# Autodesk Inventor assembly: FrameAssembly
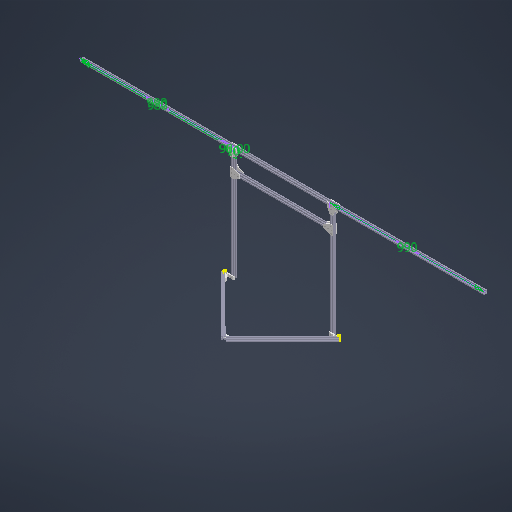
[picture p0: Inventor's stored thumbnail of the model, 512x512]
Saved by Autodesk Inventor 2026 (Build 300175050, 175E)
## iProperties
Created: 2025-06-09
Part Number: FrameAssembly
Document SubType Name: Assembly
Designer: aadit
Author: aadit
## Documents named in this file (14)
- C:\Users\aadit\OneDrive\Documents\GitHub\SWIFT-UAV\System_development\Pelican\v0.2\SubAssemblies\FrameAssembly\FrameAssembly.iam
- C:\Users\aadit\Downloads\CAD stuff\3842517173_3D_214\3842517173_3D_214\3842517173_3D_214.ipt
- C:\Users\aadit\OneDrive\Documents\GitHub\SWIFT-UAV\System_development\Pelican\v0.2\SubAssemblies\FrameAssembly\Parts\2020 T Plate Bracket Connectors .ipt
- C:\Users\aadit\OneDrive\Documents\GitHub\SWIFT-UAV\System_development\Pelican\v0.2\SubAssemblies\FrameAssembly\Parts\8020-14122\8020-14122\8020-14122.ipt
- C:\Users\aadit\OneDrive\Documents\Inventor\Content Center Files\R2026\en-US\AS 1237 (2.1)\AS 1237 - 4.ipt
- C:\Users\aadit\Documents\Inventor\Content Center Files\R2026\en-US\DIN 6912\DIN 6912 - M4 x 10.ipt
- C:\Users\aadit\OneDrive\Documents\GitHub\SWIFT-UAV\System_development\Pelican\v0.2\SubAssemblies\FrameAssembly\Parts\STRUT PROFILE 20X20 L=3100\STRUT PROFILE 20X20 L=3100\STRUT PROFILE 20X20 L=3100.ipt
- C:\Users\aadit\OneDrive\Documents\GitHub\SWIFT-UAV\System_development\Pelican\v0.2\SubAssemblies\FrameAssembly\Parts\20 Series 2 Hole - 18mm Slotted Inside Corner Bracket with Dual Support\20 Series 2 Hole - 18.ipt
- C:\Users\aadit\OneDrive\Documents\Inventor\Content Center Files\R2026\en-US\AS 1237 (2.1)\AS 1237 - 5.ipt
- C:\Users\aadit\OneDrive\Documents\Inventor\Content Center Files\R2026\en-US\DIN 6912\DIN 6912 - M5 x 16.ipt
- C:\Users\aadit\OneDrive\Documents\Inventor\Content Center Files\R2026\en-US\DIN 6912\DIN 6912 - M5 x 12.ipt
- C:\Users\aadit\OneDrive\Documents\Inventor\Content Center Files\R2026\en-US\DIN 6912\DIN 6912 - M4 x 12.ipt
- C:\Users\aadit\OneDrive\Documents\GitHub\SWIFT-UAV\System_development\Pelican\v0.2\SubAssemblies\FrameAssembly\Parts\45 Degree Connector .ipt
- C:\Users\aadit\OneDrive\Documents\GitHub\SWIFT-UAV\System_development\Pelican\v0.2\SubAssemblies\FrameAssembly\Parts\T-Nut Block\T-Nut Block\T-Nut Block.ipt
## Components (239 placed, 13 different names)
1. 3842517173_3D_214:1 — Flush:2, Mate:1, Flush:3, Flush:4, Flush:5, Flush:6, Flush:7, Flush:8, Flush:9, Flush:10, Mate:52, Mate:53, Mate:54, Mate:55
2. 3842517173_3D_214:4 — Mate:1, Flush:3, Flush:4, Flush:5, Flush:6, Flush:11, Flush:12, Flush:15, Flush:16, Mate:49, Mate:51, Mate:60, Mate:63, Mate:64
3. 3842517173_3D_214:5 — Flush:2, Flush:13, Flush:14, Flush:17, Flush:18, Mate:48, Mate:50, Mate:58, Mate:59, Mate:61, Mate:62, Mate:67
4. 2020 T Plate Bracket Connectors :1 — Flush:7, Mate:2, Mate:3, Mate:4, Mate:5, Mate:6, Insert:1, Insert:2, Insert:3, Insert:4, Insert:5, Insert:6, Insert:7, Insert:8, Insert:9, Insert:10
5. 2020 T Plate Bracket Connectors :2 — Flush:8, Mate:7, Mate:8, Mate:9, Mate:10, Mate:11, Insert:14, Insert:15, Insert:16, Insert:17, Insert:18, Insert:19, Insert:20, Insert:21, Insert:22
6. 2020 T Plate Bracket Connectors :5 — Flush:10, Mate:17, Mate:18, Mate:19, Mate:20, Mate:21, Insert:28, Insert:29, Insert:30, Insert:31, Insert:32, Insert:33, Insert:34, Insert:35, Insert:36, Insert:39
7. 2020 T Plate Bracket Connectors :8 — Flush:9, Mate:12, Mate:13, Mate:14, Mate:15, Mate:16, Mate:22, Mate:23, Mate:24, Mate:25, Mate:26, Insert:42, Insert:43, Insert:44, Insert:45, Insert:46, Insert:47, Insert:48, Insert:49, Insert:50
8. 8020-14122:1 — Mate:2
9. 8020-14122:2 — Mate:3
10. 8020-14122:3 — Mate:4
11. 8020-14122:4 — Mate:5
12. 8020-14122:5 — Mate:6
13. 8020-14122:6 — Mate:7
14. AS 1237 (2.1) 4:1 — Insert:1
15. AS 1237 (2.1) 4:2 — Insert:2
16. AS 1237 (2.1) 4:3 — Insert:3
17. AS 1237 (2.1) 4:4 — Insert:4
18. AS 1237 (2.1) 4:5 — Insert:5
19. AS 1237 (2.1) 4:6 — Insert:6, Insert:11
20. AS 1237 (2.1) 4:7 — Insert:7, Insert:12
21. AS 1237 (2.1) 4:8 — Insert:8, Insert:13
22. AS 1237 (2.1) 4:9 — Insert:9, Insert:151
23. DIN 6912 M4 x 10:1 — Insert:10
24. DIN 6912 M4 x 10:2 — Insert:11
25. DIN 6912 M4 x 10:3 — Insert:12
26. DIN 6912 M4 x 10:4 — Insert:13
27. 8020-14122:7 — Mate:8
28. 8020-14122:8 — Mate:9
29. 8020-14122:9 — Mate:10
30. 8020-14122:10 — Mate:32
31. 8020-14122:11 — Mate:11
32. AS 1237 (2.1) 4:10 — Insert:14, Insert:132
33. AS 1237 (2.1) 4:11 — Insert:15, Insert:23
34. AS 1237 (2.1) 4:12 — Insert:16
35. AS 1237 (2.1) 4:13 — Insert:17
36. AS 1237 (2.1) 4:14 — Insert:18
37. AS 1237 (2.1) 4:15 — Insert:19, Insert:24
38. AS 1237 (2.1) 4:16 — Insert:20, Insert:25
39. AS 1237 (2.1) 4:17 — Insert:21, Insert:26
40. AS 1237 (2.1) 4:18 — Insert:22, Insert:27
41. DIN 6912 M4 x 10:5 — Insert:23
42. DIN 6912 M4 x 10:6 — Insert:24
43. DIN 6912 M4 x 10:7 — Insert:25
44. DIN 6912 M4 x 10:8 — Insert:26
45. DIN 6912 M4 x 10:9 — Insert:27
46. 8020-14122:12 — Mate:12
47. 8020-14122:13 — Mate:13
48. 8020-14122:14 — Mate:14
49. 8020-14122:15 — Mate:16
50. 8020-14122:16 — Mate:15
51. 8020-14122:17 — Mate:17
52. 8020-14122:18 — Mate:19
53. 8020-14122:19 — Mate:21
54. 8020-14122:20 — Mate:18
55. 8020-14122:21 — Mate:20
56. AS 1237 (2.1) 4:19 — Insert:28, Insert:37
57. AS 1237 (2.1) 4:20 — Insert:29
58. AS 1237 (2.1) 4:21 — Insert:30
59. AS 1237 (2.1) 4:22 — Insert:31
60. AS 1237 (2.1) 4:23 — Insert:32
61. AS 1237 (2.1) 4:24 — Insert:33, Insert:38
62. AS 1237 (2.1) 4:25 — Insert:34
63. AS 1237 (2.1) 4:26 — Insert:35, Insert:40
64. AS 1237 (2.1) 4:27 — Insert:36, Insert:41
65. DIN 6912 M4 x 10:10 — Insert:37
66. DIN 6912 M4 x 10:11 — Insert:38
67. DIN 6912 M4 x 10:12 — Insert:39
68. DIN 6912 M4 x 10:13 — Insert:40
69. DIN 6912 M4 x 10:14 — Insert:41
70. 8020-14122:22 — Mate:23
71. 8020-14122:23 — Mate:22
72. 8020-14122:24 — Mate:24
73. 8020-14122:25 — Mate:25
74. 8020-14122:26 — Mate:26
75. AS 1237 (2.1) 4:28 — Insert:42, Insert:150
76. AS 1237 (2.1) 4:29 — Insert:43
77. AS 1237 (2.1) 4:30 — Insert:44
78. AS 1237 (2.1) 4:31 — Insert:45
79. AS 1237 (2.1) 4:32 — Insert:46, Insert:51
80. AS 1237 (2.1) 4:33 — Insert:47, Insert:52
81. AS 1237 (2.1) 4:34 — Insert:48, Insert:54
82. AS 1237 (2.1) 4:35 — Insert:49, Insert:53
83. AS 1237 (2.1) 4:36 — Insert:50, Insert:55
84. DIN 6912 M4 x 10:15 — Insert:51
85. DIN 6912 M4 x 10:16 — Insert:52
86. DIN 6912 M4 x 10:17 — Insert:53
87. DIN 6912 M4 x 10:18 — Insert:54
88. DIN 6912 M4 x 10:19 — Insert:55
89. STRUT PROFILE 20X20 L=3100:1 — Flush:11, Flush:12, Flush:13, Flush:14, Mate:57
90. 2020 T Plate Bracket Connectors :9 — Flush:15, Mate:43, Mate:44, Mate:45, Mate:46, Mate:47, Insert:98, Insert:99, Insert:100, Insert:101, Insert:102, Insert:103, Insert:104, Insert:105, Insert:106
91. 2020 T Plate Bracket Connectors :10 — Flush:16, Mate:33, Mate:34, Mate:35, Mate:36, Mate:37, Insert:70, Insert:71, Insert:72, Insert:73, Insert:74, Insert:75, Insert:76, Insert:77, Insert:78
92. 2020 T Plate Bracket Connectors :11 — Flush:17, Mate:38, Mate:39, Mate:40, Mate:41, Mate:42, Insert:84, Insert:85, Insert:86, Insert:87, Insert:88, Insert:89, Insert:90, Insert:91, Insert:92
93. 2020 T Plate Bracket Connectors :12 — Flush:18, Mate:27, Mate:28, Mate:29, Mate:30, Mate:31, Mate:32, Insert:56, Insert:57, Insert:58, Insert:59, Insert:60, Insert:61, Insert:62, Insert:63, Insert:64, Insert:65
94. 8020-14122:28 — Mate:27
95. 8020-14122:29 — Mate:30
96. 8020-14122:30 — Mate:28
97. 8020-14122:31 — Mate:31
98. 8020-14122:32 — Mate:29
99. 8020-14122:33 — Mate:51, Insert:126, Insert:127
100. AS 1237 (2.1) 4:37 — Insert:56
101. AS 1237 (2.1) 4:38 — Insert:57
102. AS 1237 (2.1) 4:39 — Insert:58
103. AS 1237 (2.1) 4:40 — Insert:59
104. AS 1237 (2.1) 4:41 — Insert:60
105. AS 1237 (2.1) 4:42 — Insert:61, Insert:66
106. AS 1237 (2.1) 4:43 — Insert:62, Insert:68
107. AS 1237 (2.1) 4:44 — Insert:63, Insert:67
108. AS 1237 (2.1) 4:45 — Insert:64, Insert:69
109. DIN 6912 M4 x 10:20 — Insert:65
110. DIN 6912 M4 x 10:21 — Insert:66
111. DIN 6912 M4 x 10:22 — Insert:67
112. DIN 6912 M4 x 10:23 — Insert:68
113. DIN 6912 M4 x 10:24 — Insert:69
114. 8020-14122:41 — Mate:33
115. 8020-14122:42 — Mate:35
116. 8020-14122:43 — Mate:34
117. 8020-14122:44 — Mate:36
118. 8020-14122:45 — Mate:37
119. AS 1237 (2.1) 4:46 — Insert:70, Insert:149
120. AS 1237 (2.1) 4:47 — Insert:71, Insert:79
121. AS 1237 (2.1) 4:48 — Insert:72
122. AS 1237 (2.1) 4:49 — Insert:73
123. AS 1237 (2.1) 4:50 — Insert:74
124. AS 1237 (2.1) 4:51 — Insert:75, Insert:80
125. AS 1237 (2.1) 4:52 — Insert:76, Insert:81
126. AS 1237 (2.1) 4:53 — Insert:77, Insert:82
127. AS 1237 (2.1) 4:54 — Insert:78, Insert:83
128. DIN 6912 M4 x 10:25 — Insert:79
129. DIN 6912 M4 x 10:26 — Insert:80
130. DIN 6912 M4 x 10:27 — Insert:81
131. DIN 6912 M4 x 10:28 — Insert:82
132. DIN 6912 M4 x 10:29 — Insert:83
133. 8020-14122:46 — Mate:39
134. 8020-14122:47 — Mate:40
135. 8020-14122:48 — Mate:41
136. 8020-14122:49 — Mate:42
137. 8020-14122:50 — Mate:38
138. AS 1237 (2.1) 4:55 — Insert:84, Insert:148
139. AS 1237 (2.1) 4:56 — Insert:85, Insert:93
140. AS 1237 (2.1) 4:57 — Insert:86
141. AS 1237 (2.1) 4:58 — Insert:87
142. AS 1237 (2.1) 4:59 — Insert:88
143. AS 1237 (2.1) 4:60 — Insert:89, Insert:94
144. AS 1237 (2.1) 4:61 — Insert:90, Insert:95
145. AS 1237 (2.1) 4:62 — Insert:91, Insert:96
146. AS 1237 (2.1) 4:63 — Insert:92, Insert:97
147. DIN 6912 M4 x 10:30 — Insert:93
148. DIN 6912 M4 x 10:31 — Insert:94
149. DIN 6912 M4 x 10:32 — Insert:95
150. DIN 6912 M4 x 10:33 — Insert:96
151. DIN 6912 M4 x 10:34 — Insert:97
152. 8020-14122:51 — Mate:47
153. 8020-14122:52 — Mate:43
154. 8020-14122:53 — Mate:46
155. 8020-14122:54 — Mate:44
156. 8020-14122:55 — Mate:45
157. AS 1237 (2.1) 4:64 — Insert:98, Insert:107
158. AS 1237 (2.1) 4:65 — Insert:99
159. AS 1237 (2.1) 4:66 — Insert:100
160. AS 1237 (2.1) 4:67 — Insert:101
161. AS 1237 (2.1) 4:68 — Insert:102
162. AS 1237 (2.1) 4:69 — Insert:103, Insert:108
163. AS 1237 (2.1) 4:70 — Insert:104, Insert:109
164. AS 1237 (2.1) 4:71 — Insert:105, Insert:110
165. AS 1237 (2.1) 4:72 — Insert:106, Insert:111
166. DIN 6912 M4 x 10:35 — Insert:107
167. DIN 6912 M4 x 10:36 — Insert:108
168. DIN 6912 M4 x 10:37 — Insert:109
169. DIN 6912 M4 x 10:38 — Insert:110
170. DIN 6912 M4 x 10:39 — Insert:111
171. 20 Series 2 Hole - 18:12
172. 20 Series 2 Hole - 18:14
173. 8020-14122:56 — Mate:48, Insert:112, Insert:113
174. 8020-14122:57 — Mate:49, Insert:122, Insert:123
175. 8020-14122:58 — Mate:50, Insert:118, Insert:119
176. 8020-14122:60 — Mate:52, Insert:128, Insert:129
177. 8020-14122:61 — Mate:57, Insert:139, Insert:140, Insert:146
178. 8020-14122:63 — Mate:54, Insert:116, Insert:117, Insert:120
179. 8020-14122:64 — Mate:53, Insert:114, Insert:115, Insert:134
180. 8020-14122:65 — Mate:55, Insert:124, Insert:125
181. AS 1237 (2.1) 5:1 — Insert:112, Insert:133
182. AS 1237 (2.1) 5:2 — Insert:113
183. AS 1237 (2.1) 5:3 — Insert:114
184. AS 1237 (2.1) 5:4 — Insert:115
185. AS 1237 (2.1) 5:5 — Insert:116
186. AS 1237 (2.1) 5:6 — Insert:117
187. AS 1237 (2.1) 5:7 — Insert:118
188. AS 1237 (2.1) 5:8 — Insert:119, Insert:135
189. AS 1237 (2.1) 5:9 — Insert:120, Insert:136
190. AS 1237 (2.1) 5:11 — Insert:122, Insert:147
191. AS 1237 (2.1) 5:12 — Insert:123
192. AS 1237 (2.1) 5:13 — Insert:124
193. AS 1237 (2.1) 5:14 — Insert:125, Insert:131
194. AS 1237 (2.1) 5:15 — Insert:126, Insert:137
195. AS 1237 (2.1) 5:16 — Insert:127
196. AS 1237 (2.1) 5:17 — Insert:128
197. AS 1237 (2.1) 5:18 — Insert:129, Insert:138
198. DIN 6912 M5 x 16:2 — Insert:131
199. DIN 6912 M4 x 10:40 — Insert:132
200. DIN 6912 M5 x 12:1 — Insert:133
201. DIN 6912 M4 x 12:1 — Insert:134
202. DIN 6912 M5 x 12:2 — Insert:135
203. DIN 6912 M5 x 12:3 — Insert:136
204. DIN 6912 M5 x 12:4 — Insert:137
205. DIN 6912 M5 x 12:5 — Insert:138
206. 20 Series 2 Hole - 18:16 — Mate:58
207. 8020-14122:67 — Mate:59, Insert:141, Insert:142, Insert:143, Insert:144
208. AS 1237 (2.1) 5:19 — Insert:139
209. AS 1237 (2.1) 5:20 — Insert:140
210. AS 1237 (2.1) 5:21 — Insert:141
211. AS 1237 (2.1) 5:22 — Insert:142
212. AS 1237 (2.1) 5:23 — Insert:143
213. AS 1237 (2.1) 5:24 — Insert:144, Insert:145
214. DIN 6912 M5 x 12:6 — Insert:145
215. DIN 6912 M4 x 12:2 — Insert:146
216. 20 Series 2 Hole - 18:21 — Mate:60
217. 20 Series 2 Hole - 18:22 — Mate:61
218. 20 Series 2 Hole - 18:23 — Mate:62
219. 20 Series 2 Hole - 18:24 — Mate:63
220. DIN 6912 M5 x 12:7 — Insert:147
221. DIN 6912 M4 x 10:41 — Insert:148
222. DIN 6912 M4 x 10:42 — Insert:149
223. DIN 6912 M4 x 10:43 — Insert:150
224. DIN 6912 M4 x 10:44 — Insert:151
225. 45 Degree Connector :1 — Mate:65, Mate:66, Flush:21
226. T-Nut Block:1 — Mate:64
227. T-Nut Block:3 — Mate:67
228. DIN 6912 M4 x 10:45 — Mate:65, Mate:66
229. 45 Degree Connector :2 — Insert:152, Flush:22
230. DIN 6912 M4 x 10:46 — Insert:152
231. STRUT PROFILE 20X20 L=3100:2 — Flush:21, Mate:68
232. STRUT PROFILE 20X20 L=3100:3 — Flush:22, Mate:69
233. 20 Series 2 Hole - 18:25
234. T-Nut Block:4 — Mate:68, Insert:153, Insert:154
235. T-Nut Block:5 — Mate:69, Insert:155, Insert:156
236. DIN 6912 M4 x 10:47 — Insert:153
237. DIN 6912 M4 x 10:48 — Insert:154
238. DIN 6912 M4 x 10:49 — Insert:155
239. DIN 6912 M4 x 10:50 — Insert:156
## Relationships (241: Insert 154, Mate 68, Flush 19)
- Flush:2: 3842517173_3D_214:1 ↔ 3842517173_3D_214:5
- Mate:1: 3842517173_3D_214:1 ↔ 3842517173_3D_214:4
- Flush:3: 3842517173_3D_214:1 ↔ 3842517173_3D_214:4
- Flush:4: 3842517173_3D_214:1 ↔ 3842517173_3D_214:4
- Flush:5: 3842517173_3D_214:1 ↔ 3842517173_3D_214:4
- Flush:6: 3842517173_3D_214:1 ↔ 3842517173_3D_214:4
- Flush:7: 3842517173_3D_214:1 ↔ 2020 T Plate Bracket Connectors :1
- Mate:2: 2020 T Plate Bracket Connectors :1 ↔ 8020-14122:1
- Mate:3: 2020 T Plate Bracket Connectors :1 ↔ 8020-14122:2
- Mate:4: 2020 T Plate Bracket Connectors :1 ↔ 8020-14122:3
- Mate:5: 2020 T Plate Bracket Connectors :1 ↔ 8020-14122:4
- Mate:6: 2020 T Plate Bracket Connectors :1 ↔ 8020-14122:5
- Insert:1: 2020 T Plate Bracket Connectors :1 ↔ AS 1237 (2.1) 4:1
- Insert:2: 2020 T Plate Bracket Connectors :1 ↔ AS 1237 (2.1) 4:2
- Insert:3: 2020 T Plate Bracket Connectors :1 ↔ AS 1237 (2.1) 4:3
- Insert:4: 2020 T Plate Bracket Connectors :1 ↔ AS 1237 (2.1) 4:4
- Insert:5: 2020 T Plate Bracket Connectors :1 ↔ AS 1237 (2.1) 4:5
- Insert:6: 2020 T Plate Bracket Connectors :1 ↔ AS 1237 (2.1) 4:6
- Insert:7: 2020 T Plate Bracket Connectors :1 ↔ AS 1237 (2.1) 4:7
- Insert:8: 2020 T Plate Bracket Connectors :1 ↔ AS 1237 (2.1) 4:8
- Insert:9: 2020 T Plate Bracket Connectors :1 ↔ AS 1237 (2.1) 4:9
- Insert:10: 2020 T Plate Bracket Connectors :1 ↔ DIN 6912 M4 x 10:1
- Insert:11: AS 1237 (2.1) 4:6 ↔ DIN 6912 M4 x 10:2
- Insert:12: AS 1237 (2.1) 4:7 ↔ DIN 6912 M4 x 10:3
- Insert:13: AS 1237 (2.1) 4:8 ↔ DIN 6912 M4 x 10:4
- Flush:8: 3842517173_3D_214:1 ↔ 2020 T Plate Bracket Connectors :2
- Mate:7: 2020 T Plate Bracket Connectors :2 ↔ 8020-14122:6
- Mate:8: 2020 T Plate Bracket Connectors :2 ↔ 8020-14122:7
- Mate:9: 2020 T Plate Bracket Connectors :2 ↔ 8020-14122:8
- Mate:10: 2020 T Plate Bracket Connectors :2 ↔ 8020-14122:9
- Mate:11: 2020 T Plate Bracket Connectors :2 ↔ 8020-14122:11
- Insert:14: 2020 T Plate Bracket Connectors :2 ↔ AS 1237 (2.1) 4:10
- Insert:15: 2020 T Plate Bracket Connectors :2 ↔ AS 1237 (2.1) 4:11
- Insert:16: 2020 T Plate Bracket Connectors :2 ↔ AS 1237 (2.1) 4:12
- Insert:17: 2020 T Plate Bracket Connectors :2 ↔ AS 1237 (2.1) 4:13
- Insert:18: 2020 T Plate Bracket Connectors :2 ↔ AS 1237 (2.1) 4:14
- Insert:19: 2020 T Plate Bracket Connectors :2 ↔ AS 1237 (2.1) 4:15
- Insert:20: 2020 T Plate Bracket Connectors :2 ↔ AS 1237 (2.1) 4:16
- Insert:21: 2020 T Plate Bracket Connectors :2 ↔ AS 1237 (2.1) 4:17
- Insert:22: 2020 T Plate Bracket Connectors :2 ↔ AS 1237 (2.1) 4:18
- Insert:23: AS 1237 (2.1) 4:11 ↔ DIN 6912 M4 x 10:5
- Insert:24: AS 1237 (2.1) 4:15 ↔ DIN 6912 M4 x 10:6
- Insert:25: AS 1237 (2.1) 4:16 ↔ DIN 6912 M4 x 10:7
- Insert:26: AS 1237 (2.1) 4:17 ↔ DIN 6912 M4 x 10:8
- Insert:27: AS 1237 (2.1) 4:18 ↔ DIN 6912 M4 x 10:9
- Flush:9: 3842517173_3D_214:1 ↔ 2020 T Plate Bracket Connectors :8
- Flush:10: 3842517173_3D_214:1 ↔ 2020 T Plate Bracket Connectors :5
- Mate:12: 2020 T Plate Bracket Connectors :8 ↔ 8020-14122:12
- Mate:13: 2020 T Plate Bracket Connectors :8 ↔ 8020-14122:13
- Mate:14: 2020 T Plate Bracket Connectors :8 ↔ 8020-14122:14
- Mate:15: 2020 T Plate Bracket Connectors :8 ↔ 8020-14122:16
- Mate:16: 2020 T Plate Bracket Connectors :8 ↔ 8020-14122:15
- Mate:17: 2020 T Plate Bracket Connectors :5 ↔ 8020-14122:17
- Mate:18: 2020 T Plate Bracket Connectors :5 ↔ 8020-14122:20
- Mate:19: 2020 T Plate Bracket Connectors :5 ↔ 8020-14122:18
- Mate:20: 2020 T Plate Bracket Connectors :5 ↔ 8020-14122:21
- Mate:21: 2020 T Plate Bracket Connectors :5 ↔ 8020-14122:19
- Insert:28: 2020 T Plate Bracket Connectors :5 ↔ AS 1237 (2.1) 4:19
- Insert:29: 2020 T Plate Bracket Connectors :5 ↔ AS 1237 (2.1) 4:20
- Insert:30: 2020 T Plate Bracket Connectors :5 ↔ AS 1237 (2.1) 4:21
- Insert:31: 2020 T Plate Bracket Connectors :5 ↔ AS 1237 (2.1) 4:22
- Insert:32: 2020 T Plate Bracket Connectors :5 ↔ AS 1237 (2.1) 4:23
- Insert:33: 2020 T Plate Bracket Connectors :5 ↔ AS 1237 (2.1) 4:24
- Insert:34: 2020 T Plate Bracket Connectors :5 ↔ AS 1237 (2.1) 4:25
- Insert:35: 2020 T Plate Bracket Connectors :5 ↔ AS 1237 (2.1) 4:26
- Insert:36: 2020 T Plate Bracket Connectors :5 ↔ AS 1237 (2.1) 4:27
- Insert:37: AS 1237 (2.1) 4:19 ↔ DIN 6912 M4 x 10:10
- Insert:38: AS 1237 (2.1) 4:24 ↔ DIN 6912 M4 x 10:11
- Insert:39: 2020 T Plate Bracket Connectors :5 ↔ DIN 6912 M4 x 10:12
- Insert:40: AS 1237 (2.1) 4:26 ↔ DIN 6912 M4 x 10:13
- Insert:41: AS 1237 (2.1) 4:27 ↔ DIN 6912 M4 x 10:14
- Mate:22: 2020 T Plate Bracket Connectors :8 ↔ 8020-14122:23
- Mate:23: 2020 T Plate Bracket Connectors :8 ↔ 8020-14122:22
- Mate:24: 2020 T Plate Bracket Connectors :8 ↔ 8020-14122:24
- Mate:25: 2020 T Plate Bracket Connectors :8 ↔ 8020-14122:25
- Mate:26: 2020 T Plate Bracket Connectors :8 ↔ 8020-14122:26
- Insert:42: 2020 T Plate Bracket Connectors :8 ↔ AS 1237 (2.1) 4:28
- Insert:43: 2020 T Plate Bracket Connectors :8 ↔ AS 1237 (2.1) 4:29
- Insert:44: 2020 T Plate Bracket Connectors :8 ↔ AS 1237 (2.1) 4:30
- Insert:45: 2020 T Plate Bracket Connectors :8 ↔ AS 1237 (2.1) 4:31
- Insert:46: 2020 T Plate Bracket Connectors :8 ↔ AS 1237 (2.1) 4:32
- Insert:47: 2020 T Plate Bracket Connectors :8 ↔ AS 1237 (2.1) 4:33
- Insert:48: 2020 T Plate Bracket Connectors :8 ↔ AS 1237 (2.1) 4:34
- Insert:49: 2020 T Plate Bracket Connectors :8 ↔ AS 1237 (2.1) 4:35
- Insert:50: 2020 T Plate Bracket Connectors :8 ↔ AS 1237 (2.1) 4:36
- Insert:51: AS 1237 (2.1) 4:32 ↔ DIN 6912 M4 x 10:15
- Insert:52: AS 1237 (2.1) 4:33 ↔ DIN 6912 M4 x 10:16
- Insert:53: AS 1237 (2.1) 4:35 ↔ DIN 6912 M4 x 10:17
- Insert:54: AS 1237 (2.1) 4:34 ↔ DIN 6912 M4 x 10:18
- Insert:55: AS 1237 (2.1) 4:36 ↔ DIN 6912 M4 x 10:19
- Flush:11: 3842517173_3D_214:4 ↔ STRUT PROFILE 20X20 L=3100:1
- Flush:12: 3842517173_3D_214:4 ↔ STRUT PROFILE 20X20 L=3100:1
- Flush:13: 3842517173_3D_214:5 ↔ STRUT PROFILE 20X20 L=3100:1
- Flush:14: 3842517173_3D_214:5 ↔ STRUT PROFILE 20X20 L=3100:1
- Flush:15: 3842517173_3D_214:4 ↔ 2020 T Plate Bracket Connectors :9
- Flush:16: 3842517173_3D_214:4 ↔ 2020 T Plate Bracket Connectors :10
- Flush:17: 3842517173_3D_214:5 ↔ 2020 T Plate Bracket Connectors :11
- Flush:18: 3842517173_3D_214:5 ↔ 2020 T Plate Bracket Connectors :12
- Mate:27: 2020 T Plate Bracket Connectors :12 ↔ 8020-14122:28
- Mate:28: 2020 T Plate Bracket Connectors :12 ↔ 8020-14122:30
- Mate:29: 2020 T Plate Bracket Connectors :12 ↔ 8020-14122:32
- Mate:30: 2020 T Plate Bracket Connectors :12 ↔ 8020-14122:29
- Mate:31: 2020 T Plate Bracket Connectors :12 ↔ 8020-14122:31
- Mate:32: 8020-14122:10 ↔ 2020 T Plate Bracket Connectors :12
- Insert:56: 2020 T Plate Bracket Connectors :12 ↔ AS 1237 (2.1) 4:37
- Insert:57: 2020 T Plate Bracket Connectors :12 ↔ AS 1237 (2.1) 4:38
- Insert:58: 2020 T Plate Bracket Connectors :12 ↔ AS 1237 (2.1) 4:39
- Insert:59: 2020 T Plate Bracket Connectors :12 ↔ AS 1237 (2.1) 4:40
- Insert:60: 2020 T Plate Bracket Connectors :12 ↔ AS 1237 (2.1) 4:41
- Insert:61: 2020 T Plate Bracket Connectors :12 ↔ AS 1237 (2.1) 4:42
- Insert:62: 2020 T Plate Bracket Connectors :12 ↔ AS 1237 (2.1) 4:43
- Insert:63: 2020 T Plate Bracket Connectors :12 ↔ AS 1237 (2.1) 4:44
- Insert:64: 2020 T Plate Bracket Connectors :12 ↔ AS 1237 (2.1) 4:45
- Insert:65: 2020 T Plate Bracket Connectors :12 ↔ DIN 6912 M4 x 10:20
- Insert:66: AS 1237 (2.1) 4:42 ↔ DIN 6912 M4 x 10:21
- Insert:67: AS 1237 (2.1) 4:44 ↔ DIN 6912 M4 x 10:22
- Insert:68: AS 1237 (2.1) 4:43 ↔ DIN 6912 M4 x 10:23
- Insert:69: AS 1237 (2.1) 4:45 ↔ DIN 6912 M4 x 10:24
- Mate:33: 2020 T Plate Bracket Connectors :10 ↔ 8020-14122:41
- Mate:34: 2020 T Plate Bracket Connectors :10 ↔ 8020-14122:43
- Mate:35: 2020 T Plate Bracket Connectors :10 ↔ 8020-14122:42
- Mate:36: 2020 T Plate Bracket Connectors :10 ↔ 8020-14122:44
- Mate:37: 2020 T Plate Bracket Connectors :10 ↔ 8020-14122:45
- Insert:70: 2020 T Plate Bracket Connectors :10 ↔ AS 1237 (2.1) 4:46
- Insert:71: 2020 T Plate Bracket Connectors :10 ↔ AS 1237 (2.1) 4:47
- Insert:72: 2020 T Plate Bracket Connectors :10 ↔ AS 1237 (2.1) 4:48
- Insert:73: 2020 T Plate Bracket Connectors :10 ↔ AS 1237 (2.1) 4:49
- Insert:74: 2020 T Plate Bracket Connectors :10 ↔ AS 1237 (2.1) 4:50
- Insert:75: 2020 T Plate Bracket Connectors :10 ↔ AS 1237 (2.1) 4:51
- Insert:76: 2020 T Plate Bracket Connectors :10 ↔ AS 1237 (2.1) 4:52
- Insert:77: 2020 T Plate Bracket Connectors :10 ↔ AS 1237 (2.1) 4:53
- Insert:78: 2020 T Plate Bracket Connectors :10 ↔ AS 1237 (2.1) 4:54
- Insert:79: AS 1237 (2.1) 4:47 ↔ DIN 6912 M4 x 10:25
- Insert:80: AS 1237 (2.1) 4:51 ↔ DIN 6912 M4 x 10:26
- Insert:81: AS 1237 (2.1) 4:52 ↔ DIN 6912 M4 x 10:27
- Insert:82: AS 1237 (2.1) 4:53 ↔ DIN 6912 M4 x 10:28
- Insert:83: AS 1237 (2.1) 4:54 ↔ DIN 6912 M4 x 10:29
- Mate:38: 2020 T Plate Bracket Connectors :11 ↔ 8020-14122:50
- Mate:39: 2020 T Plate Bracket Connectors :11 ↔ 8020-14122:46
- Mate:40: 2020 T Plate Bracket Connectors :11 ↔ 8020-14122:47
- Mate:41: 2020 T Plate Bracket Connectors :11 ↔ 8020-14122:48
- Mate:42: 2020 T Plate Bracket Connectors :11 ↔ 8020-14122:49
- Insert:84: 2020 T Plate Bracket Connectors :11 ↔ AS 1237 (2.1) 4:55
- Insert:85: 2020 T Plate Bracket Connectors :11 ↔ AS 1237 (2.1) 4:56
- Insert:86: 2020 T Plate Bracket Connectors :11 ↔ AS 1237 (2.1) 4:57
- Insert:87: 2020 T Plate Bracket Connectors :11 ↔ AS 1237 (2.1) 4:58
- Insert:88: 2020 T Plate Bracket Connectors :11 ↔ AS 1237 (2.1) 4:59
- Insert:89: 2020 T Plate Bracket Connectors :11 ↔ AS 1237 (2.1) 4:60
- Insert:90: 2020 T Plate Bracket Connectors :11 ↔ AS 1237 (2.1) 4:61
- Insert:91: 2020 T Plate Bracket Connectors :11 ↔ AS 1237 (2.1) 4:62
- Insert:92: 2020 T Plate Bracket Connectors :11 ↔ AS 1237 (2.1) 4:63
- Insert:93: AS 1237 (2.1) 4:56 ↔ DIN 6912 M4 x 10:30
- Insert:94: AS 1237 (2.1) 4:60 ↔ DIN 6912 M4 x 10:31
- Insert:95: AS 1237 (2.1) 4:61 ↔ DIN 6912 M4 x 10:32
- Insert:96: AS 1237 (2.1) 4:62 ↔ DIN 6912 M4 x 10:33
- Insert:97: AS 1237 (2.1) 4:63 ↔ DIN 6912 M4 x 10:34
- Mate:43: 2020 T Plate Bracket Connectors :9 ↔ 8020-14122:52
- Mate:44: 2020 T Plate Bracket Connectors :9 ↔ 8020-14122:54
- Mate:45: 2020 T Plate Bracket Connectors :9 ↔ 8020-14122:55
- Mate:46: 2020 T Plate Bracket Connectors :9 ↔ 8020-14122:53
- Mate:47: 2020 T Plate Bracket Connectors :9 ↔ 8020-14122:51
- Insert:98: 2020 T Plate Bracket Connectors :9 ↔ AS 1237 (2.1) 4:64
- Insert:99: 2020 T Plate Bracket Connectors :9 ↔ AS 1237 (2.1) 4:65
- Insert:100: 2020 T Plate Bracket Connectors :9 ↔ AS 1237 (2.1) 4:66
- Insert:101: 2020 T Plate Bracket Connectors :9 ↔ AS 1237 (2.1) 4:67
- Insert:102: 2020 T Plate Bracket Connectors :9 ↔ AS 1237 (2.1) 4:68
- Insert:103: 2020 T Plate Bracket Connectors :9 ↔ AS 1237 (2.1) 4:69
- Insert:104: 2020 T Plate Bracket Connectors :9 ↔ AS 1237 (2.1) 4:70
- Insert:105: 2020 T Plate Bracket Connectors :9 ↔ AS 1237 (2.1) 4:71
- Insert:106: 2020 T Plate Bracket Connectors :9 ↔ AS 1237 (2.1) 4:72
- Insert:107: AS 1237 (2.1) 4:64 ↔ DIN 6912 M4 x 10:35
- Insert:108: AS 1237 (2.1) 4:69 ↔ DIN 6912 M4 x 10:36
- Insert:109: AS 1237 (2.1) 4:70 ↔ DIN 6912 M4 x 10:37
- Insert:110: AS 1237 (2.1) 4:71 ↔ DIN 6912 M4 x 10:38
- Insert:111: AS 1237 (2.1) 4:72 ↔ DIN 6912 M4 x 10:39
- Mate:48: 3842517173_3D_214:5 ↔ 8020-14122:56
- Mate:49: 3842517173_3D_214:4 ↔ 8020-14122:57
- Mate:50: 3842517173_3D_214:5 ↔ 8020-14122:58
- Mate:51: 3842517173_3D_214:4 ↔ 8020-14122:33
- Mate:52: 3842517173_3D_214:1 ↔ 8020-14122:60
- Mate:53: 3842517173_3D_214:1 ↔ 8020-14122:64
- Mate:54: 3842517173_3D_214:1 ↔ 8020-14122:63
- Mate:55: 3842517173_3D_214:1 ↔ 8020-14122:65
- Insert:112: 8020-14122:56 ↔ AS 1237 (2.1) 5:1
- Insert:113: 8020-14122:56 ↔ AS 1237 (2.1) 5:2
- Insert:114: 8020-14122:64 ↔ AS 1237 (2.1) 5:3
- Insert:115: 8020-14122:64 ↔ AS 1237 (2.1) 5:4
- Insert:116: 8020-14122:63 ↔ AS 1237 (2.1) 5:5
- Insert:117: 8020-14122:63 ↔ AS 1237 (2.1) 5:6
- Insert:118: 8020-14122:58 ↔ AS 1237 (2.1) 5:7
- Insert:119: 8020-14122:58 ↔ AS 1237 (2.1) 5:8
- Insert:120: 8020-14122:63 ↔ AS 1237 (2.1) 5:9
- Insert:122: 8020-14122:57 ↔ AS 1237 (2.1) 5:11
- Insert:123: 8020-14122:57 ↔ AS 1237 (2.1) 5:12
- Insert:124: 8020-14122:65 ↔ AS 1237 (2.1) 5:13
- Insert:125: 8020-14122:65 ↔ AS 1237 (2.1) 5:14
- Insert:126: 8020-14122:33 ↔ AS 1237 (2.1) 5:15
- Insert:127: 8020-14122:33 ↔ AS 1237 (2.1) 5:16
- Insert:128: 8020-14122:60 ↔ AS 1237 (2.1) 5:17
- Insert:129: 8020-14122:60 ↔ AS 1237 (2.1) 5:18
- Insert:131: AS 1237 (2.1) 5:14 ↔ DIN 6912 M5 x 16:2
- Insert:132: AS 1237 (2.1) 4:10 ↔ DIN 6912 M4 x 10:40
- Insert:133: AS 1237 (2.1) 5:1 ↔ DIN 6912 M5 x 12:1
- Insert:134: 8020-14122:64 ↔ DIN 6912 M4 x 12:1
- Insert:135: AS 1237 (2.1) 5:8 ↔ DIN 6912 M5 x 12:2
- Insert:136: AS 1237 (2.1) 5:9 ↔ DIN 6912 M5 x 12:3
- Insert:137: AS 1237 (2.1) 5:15 ↔ DIN 6912 M5 x 12:4
- Insert:138: AS 1237 (2.1) 5:18 ↔ DIN 6912 M5 x 12:5
- Mate:57: STRUT PROFILE 20X20 L=3100:1 ↔ 8020-14122:61
- Mate:58: 3842517173_3D_214:5 ↔ 20 Series 2 Hole - 18:16
- Mate:59: 3842517173_3D_214:5 ↔ 8020-14122:67
- Insert:139: 8020-14122:61 ↔ AS 1237 (2.1) 5:19
- Insert:140: 8020-14122:61 ↔ AS 1237 (2.1) 5:20
- Insert:141: 8020-14122:67 ↔ AS 1237 (2.1) 5:21
- Insert:142: 8020-14122:67 ↔ AS 1237 (2.1) 5:22
- Insert:143: 8020-14122:67 ↔ AS 1237 (2.1) 5:23
- Insert:144: 8020-14122:67 ↔ AS 1237 (2.1) 5:24
- Insert:145: AS 1237 (2.1) 5:24 ↔ DIN 6912 M5 x 12:6
- Insert:146: 8020-14122:61 ↔ DIN 6912 M4 x 12:2
- Mate:60: 3842517173_3D_214:4 ↔ 20 Series 2 Hole - 18:21
- Mate:61: 3842517173_3D_214:5 ↔ 20 Series 2 Hole - 18:22
- Mate:62: 3842517173_3D_214:5 ↔ 20 Series 2 Hole - 18:23
- Mate:63: 3842517173_3D_214:4 ↔ 20 Series 2 Hole - 18:24
- Insert:147: AS 1237 (2.1) 5:11 ↔ DIN 6912 M5 x 12:7
- Insert:148: AS 1237 (2.1) 4:55 ↔ DIN 6912 M4 x 10:41
- Insert:149: AS 1237 (2.1) 4:46 ↔ DIN 6912 M4 x 10:42
- Insert:150: AS 1237 (2.1) 4:28 ↔ DIN 6912 M4 x 10:43
- Insert:151: AS 1237 (2.1) 4:9 ↔ DIN 6912 M4 x 10:44
- Mate:64: 3842517173_3D_214:4 ↔ T-Nut Block:1
- Mate:65: 45 Degree Connector :1 ↔ DIN 6912 M4 x 10:45
- Mate:66: 45 Degree Connector :1 ↔ DIN 6912 M4 x 10:45
- Mate:67: 3842517173_3D_214:5 ↔ T-Nut Block:3
- Insert:152: 45 Degree Connector :2 ↔ DIN 6912 M4 x 10:46
- Flush:21: 45 Degree Connector :1 ↔ STRUT PROFILE 20X20 L=3100:2
- Flush:22: 45 Degree Connector :2 ↔ STRUT PROFILE 20X20 L=3100:3
- Mate:68: STRUT PROFILE 20X20 L=3100:2 ↔ T-Nut Block:4
- Insert:153: T-Nut Block:4 ↔ DIN 6912 M4 x 10:47
- Insert:154: T-Nut Block:4 ↔ DIN 6912 M4 x 10:48
- Mate:69: STRUT PROFILE 20X20 L=3100:3 ↔ T-Nut Block:5
- Insert:155: T-Nut Block:5 ↔ DIN 6912 M4 x 10:49
- Insert:156: T-Nut Block:5 ↔ DIN 6912 M4 x 10:50
